# Autodesk Inventor assembly: Угловой v5
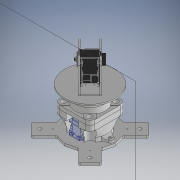
[picture p0: Inventor's stored thumbnail of the model, 180x180]
Saved by Autodesk Inventor 2022 (Build 260153000, 153)
## iProperties
Created: 2022-11-16
Part Number: Угловой v5
Document SubType Name: Assembly
Designer: Petrov Ivan
Author: Petrov Ivan
## Documents named in this file (37)
- D:\IVAN\Ivan_desktop\Kvantorium\Projects\YouBotRobot\design\Манипулятор AR\Угловой v5.iam
- D:\IVAN\Ivan_desktop\Kvantorium\Projects\YouBotRobot\design\Манипулятор AR\Днище.ipt
- D:\IVAN\Ivan_desktop\Kvantorium\Projects\YouBotRobot\design\Манипулятор AR\28Tyy.ipt
- D:\IVAN\Ivan_desktop\Kvantorium\Projects\YouBotRobot\design\Манипулятор AR\Шайба 2.ipt
- D:\IVAN\Ivan_desktop\Kvantorium\Projects\YouBotRobot\design\Манипулятор AR\Вал.ipt
- D:\IVAN\Ivan_desktop\Kvantorium\Projects\YouBotRobot\design\Манипулятор AR\Шайба1.ipt
- D:\IVAN\Ivan_desktop\Kvantorium\Projects\YouBotRobot\design\Манипулятор AR\Деталь8.ipt
- D:\IVAN\Ivan_desktop\Kvantorium\Projects\YouBotRobot\design\Манипулятор AR\snr_ucf201_0.ipt
- D:\IVAN\Ivan_desktop\Kvantorium\Projects\YouBotRobot\design\Манипулятор AR\Кожух.ipt
- D:\IVAN\Ivan_desktop\Kvantorium\Projects\YouBotRobot\design\Манипулятор AR\Стол.ipt
- D:\IVAN\Ivan_desktop\Kvantorium\Projects\YouBotRobot\design\Манипулятор AR\Сборка над столом.iam
- D:\IVAN\Ivan_desktop\Kvantorium\Projects\YouBotRobot\design\Манипулятор AR\MX-64T.ipt
- D:\IVAN\Ivan_desktop\Kvantorium\Projects\YouBotRobot\design\Манипулятор AR\Сборка длинное плечо.iam
- D:\IVAN\Ivan_desktop\Kvantorium\Projects\YouBotRobot\design\Манипулятор AR\Переходник на 64 new.ipt
- D:\IVAN\Ivan_desktop\Kvantorium\Projects\YouBotRobot\design\Манипулятор AR\Сборка среднее плечо.iam
- D:\IVAN\Ivan_desktop\Kvantorium\Projects\YouBotRobot\design\Манипулятор AR\Переходник на 28.ipt
- D:\IVAN\Ivan_desktop\Kvantorium\Projects\YouBotRobot\design\Манипулятор AR\Сборка 28 на18.iam
- D:\IVAN\Ivan_desktop\Kvantorium\Projects\YouBotRobot\design\Манипулятор AR\AX-18A.ipt
- D:\IVAN\Ivan_desktop\Kvantorium\Projects\YouBotRobot\design\Манипулятор AR\Съем1.ipt
- D:\IVAN\Ivan_desktop\Kvantorium\Projects\YouBotRobot\design\Манипулятор AR\Сборка съем.iam
- D:\IVAN\Ivan_desktop\Kvantorium\Projects\YouBotRobot\design\Манипулятор AR\Сборка клешни.iam
- D:\IVAN\Ivan_desktop\Kvantorium\Projects\YouBotRobot\design\Манипулятор AR\3d printed Gripper v4 (1).ipt
- D:\IVAN\Ivan_desktop\Kvantorium\Projects\YouBotRobot\design\Манипулятор AR\ISO 4035 - M3 - ISO.ipt
- D:\IVAN\Ivan_desktop\Kvantorium\Projects\YouBotRobot\design\Манипулятор AR\Винт M3-6gx5 ГОСТ 11738-84.ipt
- D:\IVAN\Ivan_desktop\Kvantorium\Projects\YouBotRobot\design\Манипулятор AR\ISO 4762 - M2,5 x 4ISO.ipt
- D:\IVAN\Ivan_desktop\Kvantorium\Projects\YouBotRobot\design\Манипулятор AR\ISO 4762 - M1,6 x 2,5ISO.ipt
- D:\IVAN\Ivan_desktop\Kvantorium\Projects\YouBotRobot\design\Манипулятор AR\Болт M10×1×30 ГОСТ Р 50795-95.ipt
- D:\IVAN\Ivan_desktop\Kvantorium\Projects\YouBotRobot\design\Манипулятор AR\ISO 4032 - M10 - ISO.ipt
- D:\IVAN\Ivan_desktop\Kvantorium\Projects\YouBotRobot\design\Манипулятор AR\ISO 7045 - M2,5 x 3 - 4.ipt
- D:\IVAN\Ivan_desktop\Kvantorium\Projects\YouBotRobot\design\Манипулятор AR\Винт B2.ipt
- D:\IVAN\Ivan_desktop\Kvantorium\Projects\YouBotRobot\design\Манипулятор AR\Винт B2 (1).ipt
- D:\IVAN\Ivan_desktop\Kvantorium\Projects\YouBotRobot\design\Манипулятор AR\Винт B2 (2).ipt
- D:\IVAN\Ivan_desktop\Kvantorium\Projects\YouBotRobot\design\Манипулятор AR\Гайка M2-6H ГОСТ 5929-70.ipt
- D:\IVAN\Ivan_desktop\Kvantorium\Projects\YouBotRobot\design\Манипулятор AR\Гайка M1,6-6H ГОСТ 5929-70.ipt
- D:\IVAN\Ivan_desktop\Kvantorium\Projects\YouBotRobot\design\Манипулятор AR\Гайка M1,6-6H ГОСТ 5927-70.ipt
- D:\IVAN\Ivan_desktop\Kvantorium\Projects\YouBotRobot\design\Манипулятор AR\Гайка M2,5-6H ГОСТ 5927-70.ipt
- D:\IVAN\Ivan_desktop\Kvantorium\Projects\YouBotRobot\design\Манипулятор AR\Подшипник.ipt
## Components (213 placed, 36 different names)
1. Днище:1 — Совмещение:1, Совмещение:2, Совмещение:3, Совмещение:7, Совмещение:8, Совмещение:9, Заподлицо:1, Заподлицо:2, Совмещение:19, Угол:3
2. 28Tyy:1 — Совмещение:7, Совмещение:8, Совмещение:9, Совмещение:10, Совмещение:11
3. Шайба 2:1 — Совмещение:10, Совмещение:11, Совмещение:12, Совмещение:13
4. Вал:1 — Совмещение:12, Совмещение:13, Совмещение:14, Совмещение:15
5. Шайба1:1 — Совмещение:14, Совмещение:15, Совмещение:16, Совмещение:17, Совмещение:18
6. Деталь8:1 — Совмещение:1, Совмещение:2, Совмещение:3, Совмещение:4, Совмещение:5, Совмещение:6
7. snr_ucf201_0:1 — Совмещение:4, Совмещение:5, Совмещение:6
8. Кожух:1 — Заподлицо:1, Заподлицо:2, Совмещение:19
9. Стол:1 — Совмещение:16, Совмещение:17, Совмещение:18, Совмещение:20, Совмещение:21, Совмещение:22
10. Сборка над столом:1 [sub-assembly] — Совмещение:20, Совмещение:21, Совмещение:22, Совмещение:23, Совмещение:24, Совмещение:25, Угол:2, Угол:3
11. MX-64T:1 — Совмещение:23, Совмещение:24, Совмещение:25, Совмещение:27, Совмещение:29
12. Сборка длинное плечо:1 [sub-assembly] — Заподлицо:3, Совмещение:26, Совмещение:27, Совмещение:28, Совмещение:29, Совмещение:30, Совмещение:31, Совмещение:32, Угол:2
13. Переходник на 64 new:1 — Совмещение:30, Совмещение:31, Совмещение:32, Совмещение:33, Угол:1, Угол:4
14. Сборка среднее плечо:1 [sub-assembly] — Заподлицо:4, Совмещение:34, Совмещение:35, Совмещение:36, Угол:4, Совмещение:37, Совмещение:38, Совмещение:39, Совмещение:41, Совмещение:42
15. Переходник на 28:1 — Совмещение:37, Совмещение:38, Совмещение:39, Совмещение:40
16. Сборка 28 на18:1 [sub-assembly] — Заподлицо:5, Совмещение:43, Совмещение:44, Совмещение:45, Совмещение:46, Совмещение:47, Совмещение:48
17. AX-18A:1 — Совмещение:46, Совмещение:47, Совмещение:48, Совмещение:52, Совмещение:53, Совмещение:54, Совмещение:55, Совмещение:56, Совмещение:57
18. Съем1:1 — Совмещение:49, Совмещение:50, Совмещение:51, Совмещение:52, Совмещение:53
19. Сборка съем:1 [sub-assembly] — Совмещение:56, Совмещение:57, Совмещение:58, Совмещение:59, Совмещение:60
20. Сборка клешни:1 [sub-assembly] — Совмещение:63, Совмещение:64, Угол:6
21. 3d printed Gripper v4 (1):1 — Совмещение:61, Совмещение:62, Угол:5
22. Подшипник:1 — Заподлицо:5, Совмещение:43
23. MX-64T:2 — Совмещение:28, Совмещение:33, Угол:1, Совмещение:35, Совмещение:36
24. 28Tyy:2 — Совмещение:40, Совмещение:41, Совмещение:42, Совмещение:44, Совмещение:45
25. Съем1:2 — Совмещение:49, Совмещение:50, Совмещение:51, Совмещение:54, Совмещение:55
26. AX-18A:2 — Совмещение:58, Совмещение:59, Совмещение:60, Совмещение:61, Совмещение:62, Угол:5, Совмещение:63, Совмещение:64, Угол:6
27. Кожух:2
28. Подшипник:2 — Заподлицо:4, Совмещение:34
29. Подшипник:3 — Заподлицо:3, Совмещение:26
30. ISO 4035 - M3 - ISO:2
31. Винт M3-6gx5 ГОСТ 11738-84:2
32. Винт M3-6gx5 ГОСТ 11738-84:3
33. ISO 4762 - M2,5 x 4ISO:2
34. ISO 4762 - M2,5 x 4ISO:3
35. ISO 4762 - M2,5 x 4ISO:4
36. ISO 4762 - M2,5 x 4ISO:5
37. ISO 4762 - M2,5 x 4ISO:6
38. ISO 4762 - M2,5 x 4ISO:7
39. ISO 4762 - M2,5 x 4ISO:8
40. ISO 4762 - M2,5 x 4ISO:9
41. ISO 4762 - M2,5 x 4ISO:10
42. ISO 4762 - M2,5 x 4ISO:11
43. ISO 4762 - M2,5 x 4ISO:12
44. ISO 4762 - M1,6 x 2,5ISO:2
45. ISO 4762 - M1,6 x 2,5ISO:3
46. ISO 4762 - M1,6 x 2,5ISO:4
47. ISO 4762 - M1,6 x 2,5ISO:5
48. ISO 4762 - M1,6 x 2,5ISO:6
49. ISO 4762 - M1,6 x 2,5ISO:7
50. ISO 4762 - M1,6 x 2,5ISO:8
51. ISO 4762 - M1,6 x 2,5ISO:9
52. ISO 4762 - M1,6 x 2,5ISO:10
53. ISO 4762 - M1,6 x 2,5ISO:11
54. ISO 4762 - M1,6 x 2,5ISO:12
55. ISO 4762 - M1,6 x 2,5ISO:13
56. ISO 4762 - M1,6 x 2,5ISO:14
57. ISO 4762 - M1,6 x 2,5ISO:15
58. ISO 4762 - M1,6 x 2,5ISO:16
59. ISO 4762 - M1,6 x 2,5ISO:17
60. ISO 4762 - M1,6 x 2,5ISO:18
61. ISO 4762 - M1,6 x 2,5ISO:19
62. ISO 4762 - M1,6 x 2,5ISO:20
63. ISO 4762 - M1,6 x 2,5ISO:21
64. ISO 4762 - M1,6 x 2,5ISO:22
65. ISO 4762 - M1,6 x 2,5ISO:23
66. ISO 4762 - M1,6 x 2,5ISO:24
67. ISO 4762 - M1,6 x 2,5ISO:25
68. ISO 4035 - M3 - ISO:1
69. Винт M3-6gx5 ГОСТ 11738-84:1
70. ISO 4762 - M2,5 x 4ISO:1
71. ISO 4762 - M1,6 x 2,5ISO:1
72. Болт M10×1×30 ГОСТ Р 50795-95:1
73. ISO 4032 - M10 - ISO:1
74. ISO 7045 - M2,5 x 3 - 4:1
75. Винт B2:1
76. Винт B2 (1):1
77. Винт B2 (2):1
78. Гайка M2-6H ГОСТ 5929-70:1
79. Гайка M1,6-6H ГОСТ 5929-70:1
80. Гайка M1,6-6H ГОСТ 5927-70:1
81. Гайка M2,5-6H ГОСТ 5927-70:1
82. ISO 4762 - M1,6 x 2,5ISO:26
83. ISO 4762 - M1,6 x 2,5ISO:27
84. ISO 4762 - M1,6 x 2,5ISO:28
85. ISO 4762 - M2,5 x 4ISO:13
86. ISO 4762 - M2,5 x 4ISO:14
87. Болт M10×1×30 ГОСТ Р 50795-95:2
88. Болт M10×1×30 ГОСТ Р 50795-95:3
89. Болт M10×1×30 ГОСТ Р 50795-95:4
90. ISO 4032 - M10 - ISO:2
91. ISO 4032 - M10 - ISO:3
92. ISO 4032 - M10 - ISO:4
93. ISO 7045 - M2,5 x 3 - 4:2
94. ISO 7045 - M2,5 x 3 - 4:3
95. ISO 7045 - M2,5 x 3 - 4:4
96. ISO 7045 - M2,5 x 3 - 4:5
97. ISO 7045 - M2,5 x 3 - 4:6
98. Винт B2:2
99. Винт B2:3
100. Винт B2:4
101. Винт B2:5
102. Винт B2:6
103. Винт B2:7
104. Винт B2:8
105. Винт B2 (1):2
106. Винт B2:9
107. Винт B2:10
108. Винт B2:11
109. Винт B2:12
110. Винт B2:13
111. Винт B2:14
112. Винт B2:15
113. Винт B2:16
114. Винт B2:17
115. Винт B2:18
116. Винт B2:19
117. Винт B2:20
118. Винт B2:21
119. Винт B2:22
120. Винт B2:23
121. Винт B2:24
122. Винт B2:25
123. Винт B2:26
124. Винт B2:27
125. Винт B2:28
126. Винт B2:29
127. Винт B2:30
128. Винт B2:31
129. Винт B2:32
130. Винт B2:33
131. Винт B2:34
132. Винт B2:35
133. Винт B2:36
134. Винт B2:37
135. Винт B2:38
136. Винт B2:39
137. Винт B2:40
138. Винт B2:41
139. Винт B2:42
140. Винт B2:43
141. Винт B2:44
142. Винт B2:45
143. Винт B2:46
144. Винт B2:47
145. Винт B2:48
146. Винт B2:49
147. Винт B2:50
148. Винт B2:51
149. Винт B2:52
150. Винт B2:53
151. Винт B2:54
152. Гайка M2-6H ГОСТ 5929-70:2
153. Гайка M2-6H ГОСТ 5929-70:3
154. Гайка M2-6H ГОСТ 5929-70:4
155. Гайка M2-6H ГОСТ 5929-70:5
156. Гайка M2-6H ГОСТ 5929-70:6
157. Гайка M2-6H ГОСТ 5929-70:7
158. Гайка M2-6H ГОСТ 5929-70:8
159. Гайка M2-6H ГОСТ 5929-70:9
160. Гайка M2-6H ГОСТ 5929-70:10
161. Гайка M2-6H ГОСТ 5929-70:11
162. Гайка M2-6H ГОСТ 5929-70:12
163. Гайка M2-6H ГОСТ 5929-70:13
164. Гайка M2-6H ГОСТ 5929-70:14
165. Гайка M2-6H ГОСТ 5929-70:15
166. Гайка M2-6H ГОСТ 5929-70:16
167. Гайка M2-6H ГОСТ 5929-70:17
168. Гайка M2-6H ГОСТ 5929-70:18
169. Гайка M2-6H ГОСТ 5929-70:19
170. Гайка M2-6H ГОСТ 5929-70:20
171. Гайка M1,6-6H ГОСТ 5929-70:2
172. Гайка M1,6-6H ГОСТ 5929-70:3
173. Гайка M1,6-6H ГОСТ 5929-70:4
174. Гайка M1,6-6H ГОСТ 5929-70:5
175. Гайка M2-6H ГОСТ 5929-70:21
176. Гайка M2-6H ГОСТ 5929-70:22
177. Гайка M2-6H ГОСТ 5929-70:23
178. Гайка M2-6H ГОСТ 5929-70:24
179. Гайка M1,6-6H ГОСТ 5927-70:2
180. Гайка M1,6-6H ГОСТ 5927-70:3
181. Гайка M1,6-6H ГОСТ 5927-70:4
182. Гайка M1,6-6H ГОСТ 5927-70:5
183. Гайка M1,6-6H ГОСТ 5927-70:6
184. Гайка M1,6-6H ГОСТ 5927-70:7
185. Гайка M1,6-6H ГОСТ 5927-70:8
186. Гайка M2,5-6H ГОСТ 5927-70:2
187. Гайка M2,5-6H ГОСТ 5927-70:3
188. Гайка M2,5-6H ГОСТ 5927-70:4
189. Гайка M2,5-6H ГОСТ 5927-70:5
190. Гайка M2,5-6H ГОСТ 5927-70:6
191. Гайка M2,5-6H ГОСТ 5927-70:7
192. Гайка M2,5-6H ГОСТ 5927-70:8
193. Гайка M2,5-6H ГОСТ 5927-70:9
194. Гайка M2,5-6H ГОСТ 5927-70:10
195. Гайка M2,5-6H ГОСТ 5927-70:11
196. Гайка M2,5-6H ГОСТ 5927-70:12
197. Гайка M2,5-6H ГОСТ 5927-70:13
198. Гайка M2,5-6H ГОСТ 5927-70:14
199. Гайка M2,5-6H ГОСТ 5927-70:15
200. Гайка M2,5-6H ГОСТ 5927-70:16
201. Гайка M2,5-6H ГОСТ 5927-70:17
202. Гайка M2,5-6H ГОСТ 5927-70:18
203. Гайка M2,5-6H ГОСТ 5927-70:19
204. Гайка M2,5-6H ГОСТ 5927-70:20
205. Гайка M2,5-6H ГОСТ 5927-70:21
206. Гайка M2,5-6H ГОСТ 5927-70:22
207. Гайка M2,5-6H ГОСТ 5927-70:23
208. Гайка M1,6-6H ГОСТ 5927-70:9
209. Гайка M1,6-6H ГОСТ 5927-70:10
210. Гайка M1,6-6H ГОСТ 5927-70:11
211. Гайка M1,6-6H ГОСТ 5927-70:12
212. Гайка M1,6-6H ГОСТ 5927-70:13
213. Гайка M1,6-6H ГОСТ 5927-70:14
## Relationships (75: Mate 64, Angle 6, Flush 5)
- Совмещение:1 [Mate]: Днище:1 ↔ Деталь8:1
- Совмещение:2 [Mate]: Днище:1 ↔ Деталь8:1
- Совмещение:3 [Mate]: Днище:1 ↔ Деталь8:1
- Совмещение:4 [Mate]: Деталь8:1 ↔ snr_ucf201_0:1
- Совмещение:5 [Mate]: Деталь8:1 ↔ snr_ucf201_0:1
- Совмещение:6 [Mate]: Деталь8:1 ↔ snr_ucf201_0:1
- Совмещение:7 [Mate]: Днище:1 ↔ 28Tyy:1
- Совмещение:8 [Mate]: Днище:1 ↔ 28Tyy:1
- Совмещение:9 [Mate]: Днище:1 ↔ 28Tyy:1
- Совмещение:10 [Mate] (3 mm): 28Tyy:1 ↔ Шайба 2:1
- Совмещение:11 [Mate]: 28Tyy:1 ↔ Шайба 2:1
- Совмещение:12 [Mate]: Шайба 2:1 ↔ Вал:1
- Совмещение:13 [Mate]: Шайба 2:1 ↔ Вал:1
- Совмещение:14 [Mate]: Вал:1 ↔ Шайба1:1
- Совмещение:15 [Mate]: Вал:1 ↔ Шайба1:1
- Совмещение:16 [Mate]: Шайба1:1 ↔ Стол:1
- Совмещение:17 [Mate]: Шайба1:1 ↔ Стол:1
- Совмещение:18 [Mate]: Шайба1:1 ↔ Стол:1
- Заподлицо:1 [Flush]: Днище:1 ↔ Кожух:1
- Заподлицо:2 [Flush]: Днище:1 ↔ Кожух:1
- Совмещение:19 [Mate]: Днище:1 ↔ Кожух:1
- Совмещение:20 [Mate]: Стол:1 ↔ Сборка над столом:1
- Совмещение:21 [Mate]: Стол:1 ↔ Сборка над столом:1
- Совмещение:22 [Mate]: Стол:1 ↔ Сборка над столом:1
- Совмещение:23 [Mate]: Сборка над столом:1 ↔ MX-64T:1
- Совмещение:24 [Mate]: Сборка над столом:1 ↔ MX-64T:1
- Совмещение:25 [Mate]: Сборка над столом:1 ↔ MX-64T:1
- Заподлицо:3 [Flush] (-1 mm): Сборка длинное плечо:1 ↔ Подшипник:3
- Совмещение:26 [Mate]: Сборка длинное плечо:1 ↔ Подшипник:3
- Совмещение:27 [Mate]: MX-64T:1 ↔ Сборка длинное плечо:1
- Совмещение:28 [Mate]: Сборка длинное плечо:1 ↔ MX-64T:2
- Совмещение:29 [Mate]: MX-64T:1 ↔ Сборка длинное плечо:1
- Совмещение:30 [Mate]: Сборка длинное плечо:1 ↔ Переходник на 64 new:1
- Совмещение:31 [Mate]: Сборка длинное плечо:1 ↔ Переходник на 64 new:1
- Совмещение:32 [Mate]: Сборка длинное плечо:1 ↔ Переходник на 64 new:1
- Совмещение:33 [Mate]: Переходник на 64 new:1 ↔ MX-64T:2
- Угол:1 [Angle] (0 deg): Переходник на 64 new:1 ↔ MX-64T:2
- Угол:2 [Angle] (0 deg): Сборка над столом:1 ↔ Сборка длинное плечо:1
- Угол:3 [Angle] (0 deg): Днище:1 ↔ Сборка над столом:1
- Заподлицо:4 [Flush] (-1 mm): Сборка среднее плечо:1 ↔ Подшипник:2
- Совмещение:34 [Mate]: Сборка среднее плечо:1 ↔ Подшипник:2
- Совмещение:35 [Mate]: Сборка среднее плечо:1 ↔ MX-64T:2
- Совмещение:36 [Mate]: Сборка среднее плечо:1 ↔ MX-64T:2
- Угол:4 [Angle] (0 deg): Переходник на 64 new:1 ↔ Сборка среднее плечо:1
- Совмещение:37 [Mate]: Сборка среднее плечо:1 ↔ Переходник на 28:1
- Совмещение:38 [Mate]: Сборка среднее плечо:1 ↔ Переходник на 28:1
- Совмещение:39 [Mate]: Сборка среднее плечо:1 ↔ Переходник на 28:1
- Совмещение:40 [Mate]: Переходник на 28:1 ↔ 28Tyy:2
- Совмещение:41 [Mate]: Сборка среднее плечо:1 ↔ 28Tyy:2
- Совмещение:42 [Mate]: Сборка среднее плечо:1 ↔ 28Tyy:2
- Заподлицо:5 [Flush]: Сборка 28 на18:1 ↔ Подшипник:1
- Совмещение:43 [Mate]: Сборка 28 на18:1 ↔ Подшипник:1
- Совмещение:44 [Mate]: Сборка 28 на18:1 ↔ 28Tyy:2
- Совмещение:45 [Mate]: Сборка 28 на18:1 ↔ 28Tyy:2
- Совмещение:46 [Mate]: Сборка 28 на18:1 ↔ AX-18A:1
- Совмещение:47 [Mate]: Сборка 28 на18:1 ↔ AX-18A:1
- Совмещение:48 [Mate]: Сборка 28 на18:1 ↔ AX-18A:1
- Совмещение:49 [Mate]: Съем1:1 ↔ Съем1:2
- Совмещение:50 [Mate]: Съем1:1 ↔ Съем1:2
- Совмещение:51 [Mate]: Съем1:1 ↔ Съем1:2
- Совмещение:52 [Mate]: AX-18A:1 ↔ Съем1:1
- Совмещение:53 [Mate]: AX-18A:1 ↔ Съем1:1
- Совмещение:54 [Mate]: AX-18A:1 ↔ Съем1:2
- Совмещение:55 [Mate]: AX-18A:1 ↔ Съем1:2
- Совмещение:56 [Mate]: AX-18A:1 ↔ Сборка съем:1
- Совмещение:57 [Mate]: AX-18A:1 ↔ Сборка съем:1
- Совмещение:58 [Mate]: Сборка съем:1 ↔ AX-18A:2
- Совмещение:59 [Mate]: Сборка съем:1 ↔ AX-18A:2
- Совмещение:60 [Mate]: Сборка съем:1 ↔ AX-18A:2
- Совмещение:61 [Mate]: 3d printed Gripper v4 (1):1 ↔ AX-18A:2
- Совмещение:62 [Mate]: 3d printed Gripper v4 (1):1 ↔ AX-18A:2
- Угол:5 [Angle] (179.9087 deg): 3d printed Gripper v4 (1):1 ↔ AX-18A:2
- Совмещение:63 [Mate]: Сборка клешни:1 ↔ AX-18A:2
- Совмещение:64 [Mate]: Сборка клешни:1 ↔ AX-18A:2
- Угол:6 [Angle] (0 deg): Сборка клешни:1 ↔ AX-18A:2
